# Autodesk Inventor assembly: FloorExample
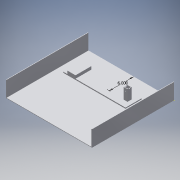
[picture p0: Inventor's stored thumbnail of the model, 180x180]
Saved by Autodesk Inventor 2016 SP1 (Build 200210100, 210)
## iProperties
Created: 2016-02-09
Part Number: FloorExample
Document SubType Name: Assembly
Designer: steele
Author: steele
## Documents named in this file (3)
- C:\snobotics\CAD-Development\robSteele\SnoBotics2016\RhinoBottomFloorOptions\FloorExample.iam
- C:\snobotics\CAD-Development\robSteele\SnoBotics2016\RhinoBottomFloorOptions\SheetBottomFloorV01.ipt
- C:\snobotics\CAD-Development\robSteele\SnoBotics2016\2016-05-05-ShooterPrototype\SupportPlateToAttachToRobotBase.ipt
## Components (2 placed, 2 different names)
1. SheetBottomFloorV01:1 — Mate:1, Mate:2, Flush:1
2. SupportPlateToAttachToRobotBase:1 — Mate:1, Mate:2, Flush:1
## Relationships (3: Mate 2, Flush 1)
- Mate:1: SheetBottomFloorV01:1 ↔ SupportPlateToAttachToRobotBase:1
- Mate:2 (101.6 mm): SheetBottomFloorV01:1 ↔ SupportPlateToAttachToRobotBase:1
- Flush:1 (-101.6 mm): SheetBottomFloorV01:1 ↔ SupportPlateToAttachToRobotBase:1
